# Autodesk Inventor assembly: TF-Luna_holder_sestava_v2
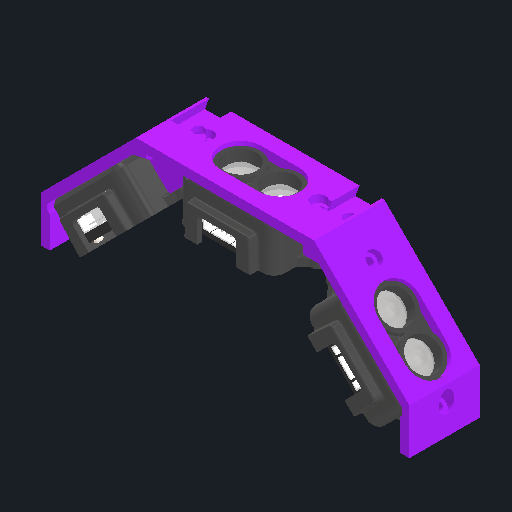
[picture p0: Inventor's stored thumbnail of the model, 512x512]
Saved by Autodesk Inventor 2025 (Build 290162000, 162)
## iProperties
Created: 2024-02-11
Part Number: TF-Luna_holder_sestava_v2
Document SubType Name: Assembly
Designer: jaryj
Author: jaryj
## Documents named in this file (3)
- C:\Users\Simak\OneDrive\Dokumenty\GitHub\RoboCop\- 3D -\_wip\TF-Luna_holder_v2\TF-Luna_holder_sestava_v2.iam
- C:\Users\Simak\OneDrive\Dokumenty\GitHub\RoboCop\- 3D -\_wip\TF-Luna_holder_v2\Držák TF-Luna.ipt
- C:\Users\Simak\OneDrive\Dokumenty\GitHub\RoboCop\- 3D -\el._parts\AssemBeneWake TF-LUNA.ipt
## Components (4 placed, 2 different names)
1. Držák TF-Luna:1 — Proti sobě:1, Proti sobě:2, Proti sobě:3, Proti sobě:4, Proti sobě:5, Proti sobě:6
2. AssemBeneWake TF-LUNA:1 — Proti sobě:1, Proti sobě:2
3. AssemBeneWake TF-LUNA:2 — Proti sobě:3, Proti sobě:4
4. AssemBeneWake TF-LUNA:3 — Proti sobě:5, Proti sobě:6
## Relationships (6: Mate 6)
- Proti sobě:1 [Mate]: Držák TF-Luna:1 ↔ AssemBeneWake TF-LUNA:1
- Proti sobě:2 [Mate]: Držák TF-Luna:1 ↔ AssemBeneWake TF-LUNA:1
- Proti sobě:3 [Mate]: Držák TF-Luna:1 ↔ AssemBeneWake TF-LUNA:2
- Proti sobě:4 [Mate]: Držák TF-Luna:1 ↔ AssemBeneWake TF-LUNA:2
- Proti sobě:5 [Mate]: Držák TF-Luna:1 ↔ AssemBeneWake TF-LUNA:3
- Proti sobě:6 [Mate]: Držák TF-Luna:1 ↔ AssemBeneWake TF-LUNA:3
